# Autodesk Inventor assembly: FinalExtruder
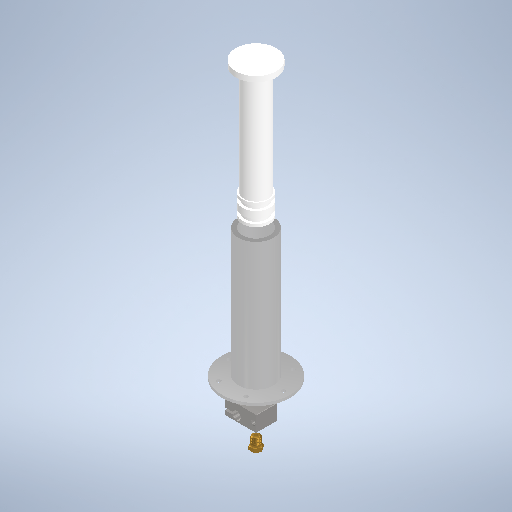
[picture p0: Inventor's stored thumbnail of the model, 512x512]
Saved by Autodesk Inventor 2025.2 (Build 292293000, 293)
## iProperties
Created: 2025-06-23
Part Number: FinalExtruder
Document SubType Name: Assembly
Designer: Simon
Author: Simon
## Documents named in this file (5)
- C:\Users\Simon\Projects\Hydrogel-3D-Printer\Hardware\Bioprinter Machine Design\Final System\Final Extruder\FinalExtruder - Copy.iam
- C:\Users\Simon\Projects\Hydrogel-3D-Printer\Hardware\Bioprinter Machine Design\PartsFolder\0.4 nozzle.ipt
- C:\Users\Simon\Projects\Hydrogel-3D-Printer\Hardware\Bioprinter Machine Design\PartsFolder\E3D-v6 Heater Block for Sensor Cartridges.ipt
- C:\Users\Simon\Projects\Hydrogel-3D-Printer\Hardware\Bioprinter Machine Design\Final System\Final Extruder\Plunger.ipt
- C:\Users\Simon\Projects\Hydrogel-3D-Printer\Hardware\Bioprinter Machine Design\Final System\Final Extruder\CylinderAttachment.ipt
## Components (4 placed, 4 different names)
1. 0.4 nozzle:1 — Mate:1, Angle:1
2. E3D-v6 Heater Block for Sensor Cartridges:1 — Mate:1, Angle:1, Mate:18
3. Plunger:1 — Mate:65
4. CylinderAttachment:1 — Mate:18, Mate:65
## Relationships (4: Mate 3, Angle 1)
- Mate:1: 0.4 nozzle:1 ↔ E3D-v6 Heater Block for Sensor Cartridges:1
- Angle:1 (0 deg): 0.4 nozzle:1 ↔ E3D-v6 Heater Block for Sensor Cartridges:1
- Mate:18: E3D-v6 Heater Block for Sensor Cartridges:1 ↔ CylinderAttachment:1
- Mate:65: Plunger:1 ↔ CylinderAttachment:1
